# Autodesk Inventor assembly: CAR_045_NewCarouselTensioner1.75UChannel
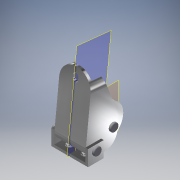
[picture p0: Inventor's stored thumbnail of the model, 180x180]
Saved by Autodesk Inventor 2018.3 (Build 223284000, 284)
## iProperties
Created: 2020-02-15
Part Number: CAR_045_NewCarouselTensioner1.75UChannel
Document SubType Name: Assembly
Designer: user
Author: user
## Documents named in this file (7)
- C:\Users\22barlalex\Documents\GrabCAD\Infinite Recharge 2020\Build season\CAR_046_NewCarouselTensioner.iam
- C:\Users\22barlalex\Documents\GrabCAD\Infinite Recharge 2020\Build season\CAR_045_NewCarouselTensioner1.75UChannel.ipt
- C:\Users\22barlalex\Documents\GrabCAD\Infinite Recharge 2020\Build season\CAR_047_98306A167_STEEL CLEVIS PIN.ipt
- C:\Users\22barlalex\Documents\GrabCAD\Infinite Recharge 2020\Build season\CAR_048_NewCarouselTensioner1.5UChannel.ipt
- C:\Users\22barlalex\Documents\GrabCAD\Infinite Recharge 2020\Build season\CAR_018_98306A167_STEEL CLEVIS PIN.ipt
- C:\Users\22barlalex\Documents\GrabCAD\Infinite Recharge 2020\Build season\CAR_014_CarouselTensionerPulley.ipt
- C:\Users\22barlalex\Documents\GrabCAD\Infinite Recharge 2020\Build season\CAR_017_57155K305_STAINLESS STEEL BALL BEARING.ipt
## Components (7 placed, 6 different names)
1. CAR_045_NewCarouselTensioner1.75UChannel:1 — Insert:1, Mate:2
2. CAR_047_98306A167_STEEL CLEVIS PIN:1 — Insert:1, Mate:1
3. CAR_048_NewCarouselTensioner1.5UChannel:1 — Mate:1, Mate:2, Insert:2, Mate:4
4. CAR_018_98306A167_STEEL CLEVIS PIN:1 — Insert:2, Mate:3
5. CAR_014_CarouselTensionerPulley:1 — Mate:3, Mate:4, Insert:3, Insert:4
6. CAR_017_57155K305_STAINLESS STEEL BALL BEARING:1 — Insert:3
7. CAR_017_57155K305_STAINLESS STEEL BALL BEARING:2 — Insert:4
## Relationships (8: Insert 4, Mate 4)
- Insert:1: CAR_045_NewCarouselTensioner1.75UChannel:1 ↔ CAR_047_98306A167_STEEL CLEVIS PIN:1
- Mate:1: CAR_047_98306A167_STEEL CLEVIS PIN:1 ↔ CAR_048_NewCarouselTensioner1.5UChannel:1
- Mate:2: CAR_045_NewCarouselTensioner1.75UChannel:1 ↔ CAR_048_NewCarouselTensioner1.5UChannel:1
- Insert:2: CAR_048_NewCarouselTensioner1.5UChannel:1 ↔ CAR_018_98306A167_STEEL CLEVIS PIN:1
- Mate:3: CAR_018_98306A167_STEEL CLEVIS PIN:1 ↔ CAR_014_CarouselTensionerPulley:1
- Mate:4: CAR_048_NewCarouselTensioner1.5UChannel:1 ↔ CAR_014_CarouselTensionerPulley:1
- Insert:3: CAR_014_CarouselTensionerPulley:1 ↔ CAR_017_57155K305_STAINLESS STEEL BALL BEARING:1
- Insert:4: CAR_014_CarouselTensionerPulley:1 ↔ CAR_017_57155K305_STAINLESS STEEL BALL BEARING:2
